# Autodesk Inventor assembly: Master Assembly V6
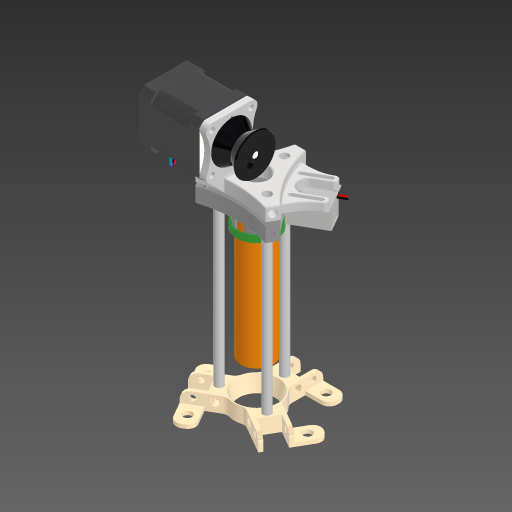
[picture p0: Inventor's stored thumbnail of the model, 512x512]
Saved by Autodesk Inventor 2024 (Build 280153000, 153)
## iProperties
Created: 2024-01-13
Part Number: Master Assembly V6
Document SubType Name: Assembly
Designer: david
Author: david
## Documents named in this file (10)
- C:\Autodesk\ChalkBot Github\ChalkbotMechanical\Chalkbot1.0\Apparatus\V6\Master Assembly V6.iam
- C:\Autodesk\ChalkBot Github\ChalkbotMechanical\Chalkbot1.0\Apparatus\V6\Top V6.ipt
- C:\Autodesk\ChalkBot Github\ChalkbotMechanical\Chalkbot1.0\Apparatus\V6\Rods.ipt
- C:\Autodesk\ChalkBot Github\ChalkbotMechanical\Chalkbot1.0\Apparatus\V6\Slider V6.ipt
- C:\Autodesk\ChalkBot Github\ChalkbotMechanical\Chalkbot1.0\Apparatus\V5\Chalk.ipt
- C:\Autodesk\ChalkBot Github\ChalkbotMechanical\Chalkbot1.0\Apparatus\V5\Stepper Pulley V14.ipt
- C:\Autodesk\ChalkBot Github\ChalkbotMechanical\Chalkbot1.0\Apparatus\V6\Collet Ring V6.ipt
- C:\Autodesk\ChalkBot Github\ChalkbotMechanical\Chalkbot1.0\Apparatus\V3\Purchased Parts\17HS19-2004S1.ipt
- C:\Autodesk\ChalkBot Github\ChalkbotMechanical\Chalkbot1.0\Apparatus\V3\Purchased Parts\Solenoid Lock.ipt
- C:\Autodesk\ChalkBot Github\ChalkbotMechanical\Chalkbot1.0\Apparatus\V6\Base V6.ipt
## Components (11 placed, 9 different names)
1. Top V6:1 — Flush:1, Flush:2, Flush:3, Mate:1, Mate:2, Mate:3, Mate:6, Mate:7, Mate:8, Mate:9, Flush:5
2. Rods:1 — Flush:1, Mate:3, Mate:4, Mate:10, Flush:6
3. Rods:2 — Flush:3, Mate:2, Mate:5, Mate:11
4. Rods:3 — Flush:2, Mate:1
5. Slider V6:1 — Mate:4, Mate:5, Insert:1, Flush:4, Cylindrical:1
6. Chalk:1 — Insert:1
7. Stepper Pulley V14:1 — Rotational:1
8. Collet Ring V6:1 — Flush:4, Cylindrical:1
9. 17HS19-2004S1:1 — Mate:6, Mate:7, Rotational:1, Mate:8
10. Solenoid Lock:1 — Mate:9, Flush:5
11. Base V6:1 — Mate:10, Flush:6, Mate:11
## Relationships (20: Mate 11, Flush 6, Insert 1, CylindricalJoint 1, RevoluteJoint 1)
- Flush:1 (5 mm): Top V6:1 ↔ Rods:1
- Flush:2 (5 mm): Top V6:1 ↔ Rods:3
- Flush:3 (5 mm): Top V6:1 ↔ Rods:2
- Mate:1: Top V6:1 ↔ Rods:3
- Mate:2: Top V6:1 ↔ Rods:2
- Mate:3: Top V6:1 ↔ Rods:1
- Mate:4: Rods:1 ↔ Slider V6:1
- Mate:5: Rods:2 ↔ Slider V6:1
- Insert:1: Slider V6:1 ↔ Chalk:1
- Flush:4: Slider V6:1 ↔ Collet Ring V6:1
- Cylindrical:1: Slider V6:1 ↔ Collet Ring V6:1
- Mate:6: Top V6:1 ↔ 17HS19-2004S1:1
- Mate:7: Top V6:1 ↔ 17HS19-2004S1:1
- Rotational:1 [RevoluteJoint]: Stepper Pulley V14:1 ↔ 17HS19-2004S1:1
- Mate:8: Top V6:1 ↔ 17HS19-2004S1:1
- Mate:9: Top V6:1 ↔ Solenoid Lock:1
- Flush:5: Top V6:1 ↔ Solenoid Lock:1
- Mate:10: Rods:1 ↔ Base V6:1
- Flush:6 (5 mm): Rods:1 ↔ Base V6:1
- Mate:11: Rods:2 ↔ Base V6:1
